# Autodesk Inventor assembly: StepperDriver_Demo_NEMA17
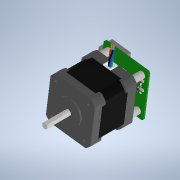
[picture p0: Inventor's stored thumbnail of the model, 180x180]
Saved by Autodesk Inventor 2022 (Build 260153000, 153)
## iProperties
Created: 2022-03-28
Part Number: StepperDriver_Demo_NEMA17
Document SubType Name: Assembly
Designer: Jorian Brusind
Author: Jorian Brusind
## Documents named in this file (5)
- C:\Users\Jorian Brusind\Documents\GitHub\HyperRail\Inventor Files\StepperDriver_Demo_NEMA17.iam
- C:\Users\Jorian Brusind\Documents\GitHub\HyperRail\Inventor Files\nema17-x-40-1.snapshot.7\NEMA17 x 40.ipt
- C:\Users\Jorian Brusind\Documents\GitHub\HyperRail\Inventor Files\Integrated Stepper Motor Driver\ExportSTEP\Main.iam
- C:\Users\Jorian Brusind\Documents\GitHub\HyperRail\Inventor Files\Metric bolt\Bolt M3 50mm.ipt
- C:\Users\Jorian Brusind\Documents\GitHub\HyperRail\Inventor Files\M3_10mmSpacer.ipt
## Components (10 placed, 4 different names)
1. NEMA17 x 40:1 — Mate:11, Mate:12, Mate:13
2. Main:1 [sub-assembly] — Mate:15
3. Bolt M3 50mm:1 — Mate:12, Mate:14
4. Bolt M3 50mm:2
5. Bolt M3 50mm:3
6. Bolt M3 50mm:4 — Mate:11
7. M3_10mmSpacer:1 — Mate:13, Flush:3, Flush:4
8. M3_10mmSpacer:2 — Flush:4, Flush:5
9. M3_10mmSpacer:3 — Flush:3
10. M3_10mmSpacer:4 — Mate:14, Flush:5, Mate:15
## Relationships (20: Mate 15, Flush 5)
- [Mate]: Main:1 ↔ M3_10mmSpacer:2
- [Mate]: Main:1 ↔ M3_10mmSpacer:1
- [Mate]: Main:1 ↔ M3_10mmSpacer:3
- [Flush]: M3_10mmSpacer:2 ↔ M3_10mmSpacer:3
- [Mate]: Main:1 ↔ Bolt M3 50mm:1
- [Mate]: Main:1 ↔ Bolt M3 50mm:2
- [Mate]: Main:1 ↔ Bolt M3 50mm:4
- [Mate]: Bolt M3 50mm:3 ↔ M3_10mmSpacer:3
- [Mate]: Main:1 ↔ Bolt M3 50mm:2
- [Mate]: Main:1 ↔ Bolt M3 50mm:1
- [Mate]: Main:1 ↔ Bolt M3 50mm:4
- [Flush]: Bolt M3 50mm:3 ↔ Bolt M3 50mm:4
- Mate:11: NEMA17 x 40:1 ↔ Bolt M3 50mm:4
- Mate:12: NEMA17 x 40:1 ↔ Bolt M3 50mm:1
- Mate:13: NEMA17 x 40:1 ↔ M3_10mmSpacer:1
- Flush:3: M3_10mmSpacer:1 ↔ M3_10mmSpacer:3
- Flush:4: M3_10mmSpacer:1 ↔ M3_10mmSpacer:2
- Mate:14: Bolt M3 50mm:1 ↔ M3_10mmSpacer:4
- Flush:5: M3_10mmSpacer:2 ↔ M3_10mmSpacer:4
- Mate:15: Main:1 ↔ M3_10mmSpacer:4
